# Autodesk Inventor assembly: under_body
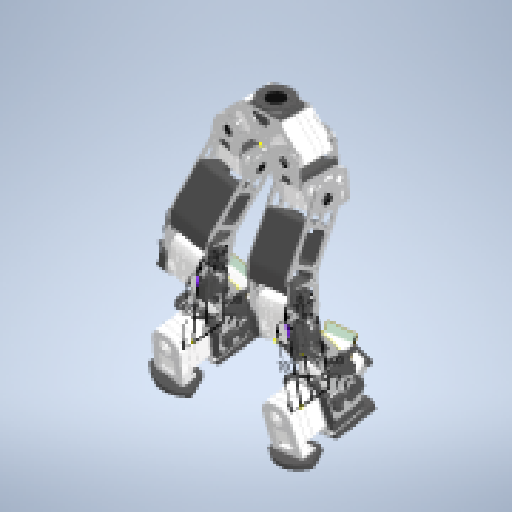
[picture p0: Inventor's stored thumbnail of the model, 512x512]
Saved by Autodesk Inventor 2024.1 (Build 281209000, 209)
## iProperties
Created: 2024-02-12
Part Number: under_body
Document SubType Name: Assembly
Designer: hibik
Author: hibik
## Documents named in this file (3)
- C:\Users\hibik\Desktop\ロボメカ\HR\2024.02.11 Rl\02.11 ProtType\under_body.iam
- C:\Users\hibik\Desktop\ロボメカ\HR\2024.02.11 Rl\02.11 ProtType\hipjoint.iam
- C:\Users\hibik\Desktop\ロボメカ\HR\2024.02.11 Rl\02.11 ProtType\leg.iam
## Components (3 placed, 2 different names)
1. hipjoint:1 [sub-assembly] — 挿入:1, 挿入:2
2. leg:1 [sub-assembly] — 挿入:1
3. leg:2 [sub-assembly] — 挿入:2
## Relationships (2: Insert 2)
- 挿入:1 [Insert]: hipjoint:1 ↔ leg:1
- 挿入:2 [Insert]: hipjoint:1 ↔ leg:2
